# Autodesk Inventor assembly: assembly_testing
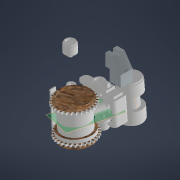
[picture p0: Inventor's stored thumbnail of the model, 180x180]
Saved by Autodesk Inventor 2022 (Build 260153000, 153)
## iProperties
Created: 2021-12-16
Part Number: assembly_testing
Document SubType Name: Assembly
Designer: MatusBarany
Author: MatusBarany
## Documents named in this file (11)
- C:\Users\Public\Documents\Autodesk\Inventor 2022\Projects\wall-e\assembly_testing.iam
- C:\Users\Public\Documents\Autodesk\Inventor 2022\Projects\wall-e\velke_koleso.ipt
- C:\Users\Public\Documents\Autodesk\Inventor 2022\Projects\wall-e\spojka_pol_velke_koleso.ipt
- C:\Users\Public\Documents\Autodesk\Inventor 2022\Projects\wall-e\stredne_koleso.ipt
- C:\Users\Public\Documents\Autodesk\Inventor 2022\Projects\wall-e\spojka_pol_stredne_koleso.ipt
- C:\Users\Public\Documents\Autodesk\Inventor 2022\Projects\wall-e\uchytka_spojky_medzi_velkym_strednym.ipt
- C:\Users\Public\Documents\Autodesk\Inventor 2022\Projects\wall-e\wheel connector.ipt
- C:\Users\Public\Documents\Autodesk\Inventor 2022\Projects\wall-e\under walle L3.ipt
- C:\Users\Public\Documents\Autodesk\Inventor 2022\Projects\wall-e\spojka_male_koleso.ipt
- C:\Users\Public\Documents\Autodesk\Inventor 2022\Projects\wall-e\male_koliesko.ipt
- C:\Users\Public\Documents\Autodesk\Inventor 2022\Projects\wall-e\chain ink.ipt
## Components (15 placed, 10 different names)
1. velke_koleso:1 — Rigid:1
2. velke_koleso:2 — Rotational:1
3. spojka_pol_velke_koleso:1 — Rotational:1, Rigid:1, Mate:1, Mate:2, Mate:3, Mate:7, Mate:8
4. stredne_koleso:1 — Rigid:2
5. stredne_koleso:2 — Rigid:3
6. spojka_pol_stredne_koleso:1 — Mate:1, Rigid:2, Rigid:3, Mate:2, Mate:3
7. uchytka_spojky_medzi_velkym_strednym:1 — Mate:4, Mate:5, Mate:6, Mate:7, Mate:8
8. wheel connector:1 — Mate:4, Mate:5, Mate:6, Rotational:2
9. under walle L3:1
10. male_koliesko:1
11. male_koliesko:2
12. male_koliesko:3 — Insert:1
13. male_koliesko:4
14. spojka_male_koleso:1 — Rotational:2, Insert:1
15. chain ink:1
## Relationships (14: Mate 8, WeldJoint 3, RevoluteJoint 2, Insert 1)
- Rotational:1 [RevoluteJoint]: velke_koleso:2 ↔ spojka_pol_velke_koleso:1
- Rigid:1 [WeldJoint]: velke_koleso:1 ↔ spojka_pol_velke_koleso:1
- Mate:1: spojka_pol_velke_koleso:1 ↔ spojka_pol_stredne_koleso:1
- Rigid:2 [WeldJoint]: stredne_koleso:1 ↔ spojka_pol_stredne_koleso:1
- Rigid:3 [WeldJoint]: stredne_koleso:2 ↔ spojka_pol_stredne_koleso:1
- Mate:2: spojka_pol_velke_koleso:1 ↔ spojka_pol_stredne_koleso:1
- Mate:3: spojka_pol_velke_koleso:1 ↔ spojka_pol_stredne_koleso:1
- Mate:4: uchytka_spojky_medzi_velkym_strednym:1 ↔ wheel connector:1
- Mate:5: uchytka_spojky_medzi_velkym_strednym:1 ↔ wheel connector:1
- Mate:6: uchytka_spojky_medzi_velkym_strednym:1 ↔ wheel connector:1
- Rotational:2 [RevoluteJoint]: wheel connector:1 ↔ spojka_male_koleso:1
- Mate:7: spojka_pol_velke_koleso:1 ↔ uchytka_spojky_medzi_velkym_strednym:1
- Mate:8: spojka_pol_velke_koleso:1 ↔ uchytka_spojky_medzi_velkym_strednym:1
- Insert:1: male_koliesko:3 ↔ spojka_male_koleso:1
